# Autodesk Inventor assembly: Coupler lift bottom fixed + pulleys
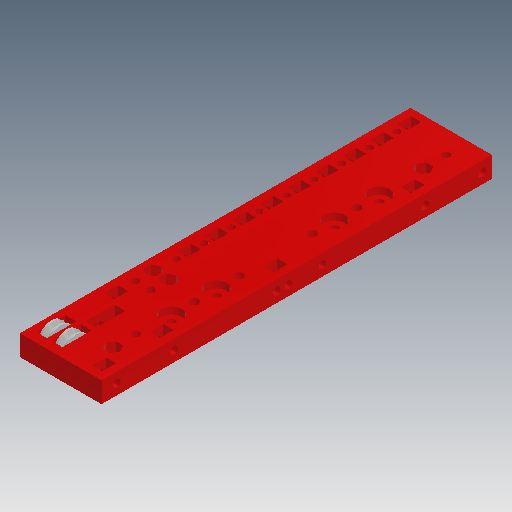
[picture p0: Inventor's stored thumbnail of the model, 512x512]
Saved by Autodesk Inventor 2020 (Build 240168000, 168)
## iProperties
Created: 2019-11-24
Part Number: Coupler lift bottom fixed + pulleys
Document SubType Name: Assembly
Designer: ball
Author: ball
## Documents named in this file (3)
- C:\FTC\FTC8863CAD\2019 Robot\Delivery\Old\Coupler lift bottom fixed + pulleys.iam
- C:\FTC\FTC8863CAD\2019 Robot\Delivery\Old\Coupler lift long.ipt
- C:\FTC\FTC8863CAD\RevRobotics\REV-41-1368 pulley.ipt
## Components (3 placed, 2 different names)
1. Coupler lift long:1 — Mate:1, Flush:1, Mate:2, Mate:3
2. REV-41-1368 pulley:1 — Mate:1, Flush:1
3. REV-41-1368 pulley:2 — Mate:2, Mate:3
## Relationships (4: Mate 3, Flush 1)
- Mate:1: Coupler lift long:1 ↔ REV-41-1368 pulley:1
- Flush:1: Coupler lift long:1 ↔ REV-41-1368 pulley:1
- Mate:2: Coupler lift long:1 ↔ REV-41-1368 pulley:2
- Mate:3: Coupler lift long:1 ↔ REV-41-1368 pulley:2
